# Autodesk Inventor assembly: Assembly1
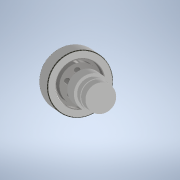
[picture p0: Inventor's stored thumbnail of the model, 180x180]
Saved by Autodesk Inventor 2021 (Build 250183000, 183)
## iProperties
Created: 2021-07-15
Part Number: Assembly1
Document SubType Name: Assembly
Designer: HP
Author: HP
## Documents named in this file (4)
- F:\Autodesk Invo\MII\Assembly1.iam
- F:\Autodesk Invo\MII\wheel.ipt
- F:\Autodesk Invo\MII\DC.ipt
- F:\Autodesk Invo\MII\Dc catcher.ipt
## Components (3 placed, 3 different names)
1. wheel:1 — Mate:6, Mate:7
2. DC:1 — Mate:3, Mate:4, Rigid:1, Mate:6, Mate:7
3. Dc catcher:1 — Mate:3, Mate:4, Rigid:1
## Relationships (5: Mate 4, WeldJoint 1)
- Mate:3: DC:1 ↔ Dc catcher:1
- Mate:4: DC:1 ↔ Dc catcher:1
- Rigid:1 [WeldJoint]: DC:1 ↔ Dc catcher:1
- Mate:6 (5 mm): wheel:1 ↔ DC:1
- Mate:7: wheel:1 ↔ DC:1
